# Autodesk Inventor assembly: head-assembled
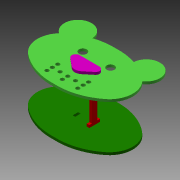
[picture p0: Inventor's stored thumbnail of the model, 180x180]
Saved by Autodesk Inventor 2013 (Build 170138000, 138)
## iProperties
Created: 2012-09-15
Part Number: head-assembled
Document SubType Name: Assembly
Designer: frankenteddy
Author: frankenteddy
## Documents named in this file (5)
- C:\Users\frankenteddy\Desktop\oshawatt1\head-assembled.iam
- C:\Users\frankenteddy\Desktop\oshawatt1\head-back.ipt
- C:\Users\frankenteddy\Desktop\oshawatt1\head-strut.ipt
- C:\Users\frankenteddy\Desktop\oshawatt1\head-front.ipt
- C:\Users\frankenteddy\Desktop\oshawatt1\head-nose.ipt
## Components (4 placed, 4 different names)
1. head-back:1 — Mate:1, Mate:2, Mate:3
2. head-strut:1 — Mate:1, Mate:2, Mate:3
3. head-front:1
4. head-nose:1
## Relationships (3: Mate 3)
- Mate:1: head-back:1 ↔ head-strut:1
- Mate:2: head-back:1 ↔ head-strut:1
- Mate:3: head-back:1 ↔ head-strut:1
